# Autodesk Inventor assembly: Cylinder, Air Push, Spring Return
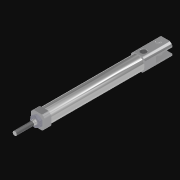
[picture p0: Inventor's stored thumbnail of the model, 180x180]
Saved by Autodesk Inventor 2021 (Build 250183000, 183)
## iProperties
Created: 2011-03-21
Part Number: Cylinder, Air Push, Spring Return
Document SubType Name: Assembly
Designer: Jordan
Mass: 9.12115 g
Surface Area: 87.2403 cm^2
Volume: 9.12115 cm^3
Density: 1 g/cm^3
Translation Standard: STEP AP203
FileName: Cylinder, Air Push, Spring Return.iam
PreProcessor: SolidWorks 2011
PostProcessor: Build: 239, Release: 2011 RTM - Date: Wed 02/17/2010
Sent Units: millimeter
Uncertainty: 1e-05
Author: Jordan
## Documents named in this file (4)
- E:\VEX Library\Motion\Pneumatics\Cylinder, Air Push, Spring Return.iam
- E:\VEX Library\Structure\Hardware\Nut M5 Thin Hex.ipt
- E:\VEX Library\Motion\Pneumatics\Reference Parts\Cylinder, Air Push, Spring Return\Body.ipt
- E:\VEX Library\Motion\Pneumatics\Reference Parts\Cylinder, Air Push, Spring Return\Rod.ipt
## Components (3 placed, 3 different names)
1. Nut M5 Thin Hex:1 — Angle:1
2. Body:1
3. Rod:1 — Angle:1
## Relationships (1: Angle 1)
- Angle:1 (0 deg): Nut M5 Thin Hex:1 ↔ Rod:1
